# Autodesk Inventor assembly: samenstelling
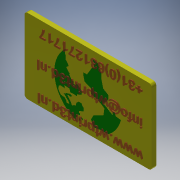
[picture p0: Inventor's stored thumbnail of the model, 180x180]
Saved by Autodesk Inventor 2019 (Build 230136000, 136)
## iProperties
Created: 2020-06-08
Part Number: samenstelling
Document SubType Name: Assembly
Designer: Jaap Kort
Author: Jaap Kort
## Documents named in this file (4)
- C:\Users\windo\Desktop\visitekaartje\samenstelling.iam
- C:\Users\windo\Desktop\visitekaartje\kaart.ipt
- C:\Users\windo\Desktop\visitekaartje\aarde.ipt
- C:\Users\windo\Desktop\visitekaartje\tekst.ipt
## Components (3 placed, 3 different names)
1. kaart:1 — Flush:1, Mate:1, Flush:2, Mate:2, Mate:3, Mate:4
2. aarde:1 — Flush:1, Mate:1, Flush:2
3. tekst:1 — Mate:2, Mate:3, Mate:4
## Relationships (6: Mate 4, Flush 2)
- Flush:1: kaart:1 ↔ aarde:1
- Mate:1 (-42.5 mm): kaart:1 ↔ aarde:1
- Flush:2 (-25 mm): kaart:1 ↔ aarde:1
- Mate:2: kaart:1 ↔ tekst:1
- Mate:3: kaart:1 ↔ tekst:1
- Mate:4: kaart:1 ↔ tekst:1
